# Autodesk Inventor assembly: Base_Assembly
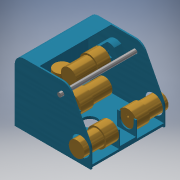
[picture p0: Inventor's stored thumbnail of the model, 180x180]
Saved by Autodesk Inventor 2016 (Build 200138000, 138)
## iProperties
Created: 2015-05-19
Part Number: Base_Assembly
Document SubType Name: Assembly
Designer: CHUNGBK
Author: CHUNGBK
## Documents named in this file (4)
- C:\Users\jonathan\Desktop\Five Axis Serial Robotic Arm\Inventor\Scorbot Platform.iam
- C:\Users\jonathan\Desktop\Five Axis Serial Robotic Arm\Inventor\Platform Link.ipt
- C:\Users\jonathan\Desktop\Five Axis Serial Robotic Arm\Inventor\Motor.ipt
- C:\Users\jonathan\Desktop\Five Axis Serial Robotic Arm\Inventor\Platform Rod.ipt
## Components (7 placed, 3 different names)
1. Platform Link:1 — Flush:2, Flush:1, Flush:3, Mate:1, Mate:2, Mate:4, Mate:5, Mate:6, Mate:7, Mate:8, Mate:9, Mate:10, Mate:11, Flush:4, Mate:12, Angle:1, Angle:2, Mate:13, Mate:14, Angle:3
2. Motor:1 — Mate:1, Mate:2, Angle:1
3. Motor:2 — Mate:7, Mate:8, Mate:13
4. Motor:3 — Mate:9, Mate:10, Mate:14
5. Motor:4 — Mate:4, Mate:12, Angle:2
6. Motor:5 — Mate:5, Mate:6, Angle:3
7. Platform Rod:1 — Mate:11, Flush:4
## Relationships (20: Mate 13, Flush 4, Angle 3)
- Flush:2: Platform Link:1
- Flush:1: Platform Link:1
- Flush:3: Platform Link:1
- Mate:1: Platform Link:1 ↔ Motor:1
- Mate:2: Platform Link:1 ↔ Motor:1
- Mate:4: Platform Link:1 ↔ Motor:4
- Mate:5: Platform Link:1 ↔ Motor:5
- Mate:6: Platform Link:1 ↔ Motor:5
- Mate:7: Platform Link:1 ↔ Motor:2
- Mate:8 (38.1 mm): Platform Link:1 ↔ Motor:2
- Mate:9: Platform Link:1 ↔ Motor:3
- Mate:10 (38.1 mm): Platform Link:1 ↔ Motor:3
- Mate:11: Platform Link:1 ↔ Platform Rod:1
- Flush:4 (-7.3025 mm): Platform Link:1 ↔ Platform Rod:1
- Mate:12: Platform Link:1 ↔ Motor:4
- Angle:1 (180 deg): Platform Link:1 ↔ Motor:1
- Angle:2 (0 deg): Platform Link:1 ↔ Motor:4
- Mate:13: Platform Link:1 ↔ Motor:2
- Mate:14: Platform Link:1 ↔ Motor:3
- Angle:3 (0 deg): Platform Link:1 ↔ Motor:5
